# Autodesk Inventor assembly: Assembly3
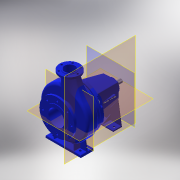
[picture p0: Inventor's stored thumbnail of the model, 180x180]
Saved by Autodesk Inventor 2016 (Build 200138000, 138)
## iProperties
Created: 2017-06-07
Part Number: Assembly3
Document SubType Name: Assembly
Designer: Mohamed
Author: Mohamed
## Documents named in this file (3)
- C:\Users\Mohamed\Desktop\Assembly3.iam
- C:\Users\Mohamed\Desktop\pump.ipt
- C:\Users\Mohamed\Desktop\DIN 933 - M14  x 16.ipt
## Components (7 placed, 2 different names)
1. pump:1 — Mate:1, Mate:2, Mate:3, Mate:4, Flush:1
2. DIN 933 - M14  x 16:1 — Mate:1, Mate:2
3. DIN 933 - M14  x 16:2
4. DIN 933 - M14  x 16:3
5. DIN 933 - M14  x 16:4
6. DIN 933 - M14  x 16:5
7. DIN 933 - M14  x 16:6
## Component patterns: (6 elements, first: DIN 933 - M14  x 16:1)
## Relationships (5: Mate 4, Flush 1)
- Mate:1: pump:1 ↔ DIN 933 - M14  x 16:1
- Mate:2: pump:1 ↔ DIN 933 - M14  x 16:1
- Mate:3: pump:1
- Mate:4: pump:1
- Flush:1: pump:1
